# Autodesk Inventor assembly: Screw_Sub
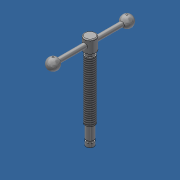
[picture p0: Inventor's stored thumbnail of the model, 180x180]
Saved by Autodesk Inventor 2022.4 (Build 264492010, 492A)
## iProperties
Created: 2006-01-18
Part Number: Screw_Sub
Document SubType Name: Assembly
Designer: PMiller
Author: PMiller
## iProperties of the stored document MemberDocs/xNvseamhpAsjbdovqB2itnhvfUa
Created: 2006-01-18
Part Number: Screw_Sub
Document SubType Name: Assembly
Designer: PMiller
Mass: 357.514 g
Surface Area: 166.374 cm^2
Volume: 45.5432 cm^3
Density: 7.85 g/cm^3
Author: PMiller
## iProperties of the stored document MemberDocs/xCdzpukv3HcmgoukbPznnhzifYf
Created: 2006-01-18
Part Number: Screw_Sub
Document SubType Name: Assembly
Designer: PMiller
Mass: 295.363 g
Surface Area: 146.425 cm^2
Volume: 37.6259 cm^3
Density: 7.85 g/cm^3
Author: PMiller
## Documents named in this file (5)
- U:\Inventor 2022 Training\_Designer Training\Inventor 2022 - Advanced Assembly\Practice Files\Model States\Screw_Sub_Model_States.iam
- U:\Inventor 2022 Training\_Designer Training\Inventor 2022 - Advanced Assembly\Practice Files\Model States\Vise_Screw_Model_States.ipt
- U:\Inventor 2022 Training\_Designer Training\Inventor 2022 - Advanced Assembly\Practice Files\Model States\Handle_Rod.ipt
- U:\Inventor 2022 Training\_Designer Training\Inventor 2022 - Advanced Assembly\Practice Files\Model States\Handle_Ball.ipt
- U:\Inventor 2022 Training\_Designer Training\Inventor 2022 - Advanced Assembly\Practice Files\Model States\Pin.ipt
## Components (6 placed, 4 different names)
1. Vise_Screw_Model_States:1 — Mate:7, Mate:8
2. Handle_Rod:1 — Mate:1, Mate:2, Mate:3, Mate:4, Mate:5, Mate:6, Mate:7, Mate:8
3. Handle_Ball:1 — Mate:4, Mate:5, Mate:6, Insert:1
4. Handle_Ball:2 — Mate:1, Mate:2, Mate:3, Insert:2
5. Pin:1 — Insert:1
6. Pin:2 — Insert:2
## Relationships (10: Mate 8, Insert 2)
- Mate:1: Handle_Rod:1 ↔ Handle_Ball:2
- Mate:2: Handle_Rod:1 ↔ Handle_Ball:2
- Mate:3: Handle_Rod:1 ↔ Handle_Ball:2
- Mate:4: Handle_Rod:1 ↔ Handle_Ball:1
- Mate:5: Handle_Rod:1 ↔ Handle_Ball:1
- Mate:6: Handle_Rod:1 ↔ Handle_Ball:1
- Insert:1: Handle_Ball:1 ↔ Pin:1
- Insert:2: Handle_Ball:2 ↔ Pin:2
- Mate:7: Vise_Screw_Model_States:1 ↔ Handle_Rod:1
- Mate:8: Vise_Screw_Model_States:1 ↔ Handle_Rod:1
